# Autodesk Inventor assembly: Winch mount assenbly
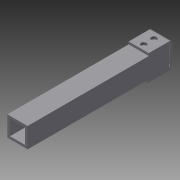
[picture p0: Inventor's stored thumbnail of the model, 180x180]
Saved by Autodesk Inventor 2013 (Build 170138000, 138)
## iProperties
Created: 2013-02-03
Part Number: Winch mount assenbly
Document SubType Name: Assembly
Designer: Arpan
Author: Arpan
## Documents named in this file (3)
- C:\Users\Arpan\Documents\GitHub\frc2013CAD\Cimber actual\Winch mount assenbly.iam
- C:\Users\Arpan\Documents\GitHub\frc2013CAD\Cimber actual\winch mount.ipt
- C:\Users\Arpan\Documents\GitHub\frc2013CAD\Cimber actual\Winch mount frange.ipt
## Components (2 placed, 2 different names)
1. winch mount:1 — Mate:1, Mate:2, Flush:1
2. Winch mount frange:1 — Mate:1, Mate:2, Flush:1
## Relationships (3: Mate 2, Flush 1)
- Mate:1: winch mount:1 ↔ Winch mount frange:1
- Mate:2: winch mount:1 ↔ Winch mount frange:1
- Flush:1: winch mount:1 ↔ Winch mount frange:1
